# Autodesk Inventor assembly: xShaft
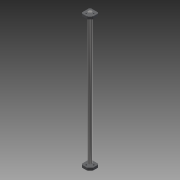
[picture p0: Inventor's stored thumbnail of the model, 180x180]
Saved by Autodesk Inventor 2013 (Build 170138000, 138)
## iProperties
Created: 2015-01-14
Part Number: xShaft
Document SubType Name: Assembly
Designer: dzban
Author: dzban
## Documents named in this file (3)
- D:\PIRX\Artisan\OPENSOURCE\SmallPieces\xShaft.iam
- D:\PIRX\Artisan\OPENSOURCE\SmallPieces\xShaftHolder.ipt
- D:\PIRX\Artisan\OPENSOURCE\XCars\Xshaft.ipt
## Components (3 placed, 2 different names)
1. xShaftHolder:1 — Insert:2, Flush:1
2. xShaftHolder:2 — Insert:1, Flush:1
3. Xshaft:1 — Insert:1, Insert:2
## Relationships (3: Insert 2, Flush 1)
- Insert:1 (-6 mm): xShaftHolder:2 ↔ Xshaft:1
- Insert:2 (-6 mm): xShaftHolder:1 ↔ Xshaft:1
- Flush:1: xShaftHolder:1 ↔ xShaftHolder:2
